# Autodesk Inventor assembly: VacuumTubeHolder
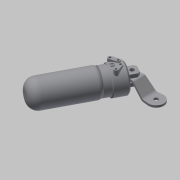
[picture p0: Inventor's stored thumbnail of the model, 180x180]
Saved by Autodesk Inventor 2015 SP1 (Build 190203100, 203)
## iProperties
Created: 2015-06-28
Part Number: VacuumTubeHolder
Document SubType Name: Assembly
Designer: Val
Author: Val
## Documents named in this file (4)
- C:\Users\Val\Desktop\ExoGit\elysium-max-exoskeleton\src\Assemblies\VacuumTubeHolder.iam
- C:\Users\Val\Desktop\ExoGit\elysium-max-exoskeleton\src\BackConnector.ipt
- C:\Users\Val\Desktop\ExoGit\elysium-max-exoskeleton\src\VacuumTubeHolderBase.ipt
- C:\Users\Val\Desktop\ExoGit\elysium-max-exoskeleton\src\External\VacuumTube6L6GCSTR440.ipt
## Components (3 placed, 3 different names)
1. BackConnector:1 — Mate:1, Mate:2
2. VacuumTubeHolderBase:1 — Mate:1, Mate:2, Mate:3, Mate:4
3. VacuumTube:1 — Mate:3, Mate:4
## Relationships (4: Mate 4)
- Mate:1: BackConnector:1 ↔ VacuumTubeHolderBase:1
- Mate:2: BackConnector:1 ↔ VacuumTubeHolderBase:1
- Mate:3 (-6.5 mm): VacuumTubeHolderBase:1 ↔ VacuumTube:1
- Mate:4: VacuumTubeHolderBase:1 ↔ VacuumTube:1
